# Autodesk Inventor assembly: buttons
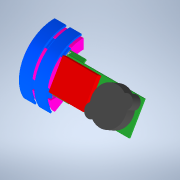
[picture p0: Inventor's stored thumbnail of the model, 180x180]
Saved by Autodesk Inventor 2020 (Build 240168000, 168)
## iProperties
Created: 2019-11-15
Part Number: buttons
Document SubType Name: Assembly
Designer: suchanek
Author: suchanek
## Documents named in this file (7)
- D:\suchanek\programming\rowing_steering\model_final\buttons1.iam
- D:\suchanek\programming\rowing_steering\model_final\export\Workspaces\Workspace\buttons_push_button.ipt
- D:\suchanek\programming\rowing_steering\model_final\export\Workspaces\Workspace\buttons_base.ipt
- D:\suchanek\programming\rowing_steering\model_final\export\Workspaces\Workspace\buttons_button_cap.ipt
- D:\suchanek\programming\rowing_steering\model_final\buttons_battery.ipt
- D:\suchanek\programming\rowing_steering\model_final\buttons_BLE_nano.ipt
- D:\suchanek\programming\rowing_steering\model_final\buttons1_PCBs.ipt
## Components (10 placed, 6 different names)
1. buttons_push_button:1 — Slider:1, Symmetry:2
2. buttons_base:1 — Slider:1, Slider:2, Slider:3, Slider:4, Flush:2, Cylindrical:1, Mate:1, Flush:3, Mate:4, Mate:5, Mate:6, Mate:7
3. buttons_push_button:2 — Slider:2, Flush:1, Symmetry:2
4. buttons_push_button:3 — Slider:3, Symmetry:1
5. buttons_push_button:4 — Slider:4, Flush:1, Symmetry:1
6. buttons_button_cap:1 — Cylindrical:1, Mate:1, Flush:3, Mate:2, Flush:4, Symmetry:3
7. buttons_button_cap:2 — Mate:2, Flush:4, Symmetry:3
8. buttons_battery:1 — Mate:3, Tangent:1, Tangent:2
9. buttons_BLE_nano:1 — Slider:5, Mate:4
10. buttons1_PCBs:1 — Slider:5, Mate:3, Tangent:1, Tangent:2, Mate:5, Mate:6, Mate:7
## Relationships (22: Mate 7, TranslationJoint 5, Flush 4, Symmetry 3, Tangent 2, CylindricalJoint 1)
- Slider:1 [TranslationJoint] (1 mm): buttons_push_button:1 ↔ buttons_base:1
- Slider:2 [TranslationJoint] (1 mm): buttons_base:1 ↔ buttons_push_button:2
- Slider:3 [TranslationJoint] (1 mm): buttons_base:1 ↔ buttons_push_button:3
- Slider:4 [TranslationJoint] (1 mm): buttons_base:1 ↔ buttons_push_button:4
- Flush:1: buttons_push_button:2 ↔ buttons_push_button:4
- Flush:2 (-10 mm): buttons_base:1
- Symmetry:1: buttons_push_button:3 ↔ buttons_push_button:4
- Symmetry:2: buttons_push_button:1 ↔ buttons_push_button:2
- Cylindrical:1: buttons_base:1 ↔ buttons_button_cap:1
- Mate:1 (0.35 mm): buttons_base:1 ↔ buttons_button_cap:1
- Flush:3: buttons_base:1 ↔ buttons_button_cap:1
- Mate:2: buttons_button_cap:1 ↔ buttons_button_cap:2
- Flush:4: buttons_button_cap:1 ↔ buttons_button_cap:2
- Symmetry:3: buttons_button_cap:1 ↔ buttons_button_cap:2
- Slider:5 [TranslationJoint]: buttons_BLE_nano:1 ↔ buttons1_PCBs:1
- Mate:3: buttons_battery:1 ↔ buttons1_PCBs:1
- Tangent:1: buttons_battery:1 ↔ buttons1_PCBs:1
- Tangent:2: buttons_battery:1 ↔ buttons1_PCBs:1
- Mate:4: buttons_base:1 ↔ buttons_BLE_nano:1
- Mate:5: buttons_base:1 ↔ buttons1_PCBs:1
- Mate:6: buttons_base:1 ↔ buttons1_PCBs:1
- Mate:7: buttons_base:1 ↔ buttons1_PCBs:1
